# Autodesk Inventor assembly: daVinciHead_HITEC_Assembly
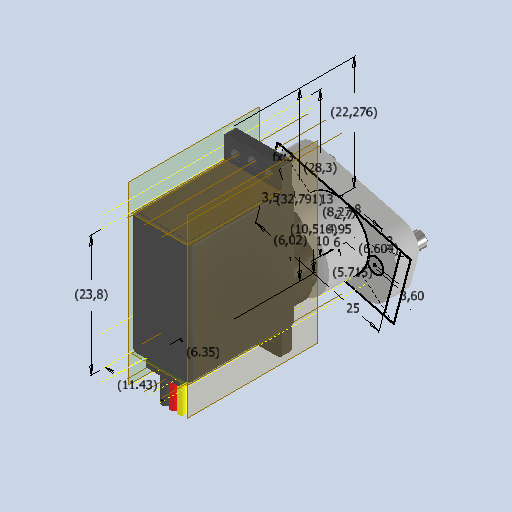
[picture p0: Inventor's stored thumbnail of the model, 512x512]
Saved by Autodesk Inventor 2024 (Build 280153000, 153)
## iProperties
Created: 2022-08-20
Part Number: daVinciHead_HITEC_Assembly
Document SubType Name: Assembly
Designer: alexw
Mass: 9.99183 g
Surface Area: 44.3615 cm^2
Volume: 8.83133 cm^3
Author: alexw
## Documents named in this file (6)
- C:\Users\AEWALDER\Documents\Inventor\03_CurrentProjects\MasterThesis\PSM_V1_Rillenkugellager\Ueberarbeiteter DaVincikopf\daVinciHead_HITEC_Assembly.iam
- C:\Users\AEWALDER\Documents\Inventor\03_CurrentProjects\MasterThesis\PSM_V1_Rillenkugellager\Ueberarbeiteter DaVincikopf\Hitec HS-65HB.ipt
- C:\Users\AEWALDER\Documents\Inventor\03_CurrentProjects\MasterThesis\PSM_V1_Rillenkugellager\Ueberarbeiteter DaVincikopf\daVinci_Tool_Clutch.ipt
- C:\Users\AEWALDER\Documents\Inventor\03_CurrentProjects\MasterThesis\PSM_V1_Rillenkugellager\Ueberarbeiteter DaVincikopf\daVinci_Tool_Clutch_Pins.ipt
- C:\Users\AEWALDER\Documents\Inventor\03_CurrentProjects\MasterThesis\PSM_V1_Rillenkugellager\ContentCenter\de-DE\ISO 4762(2)\ISO 4762 - M2 x 5ISO.ipt
- C:\Users\AEWALDER\Documents\Inventor\03_CurrentProjects\MasterThesis\PSM_V1_Rillenkugellager\ContentCenter\de-DE\ISO 7089\ISO 7089 - 2 - 140 HV(1).ipt
## Components (6 placed, 5 different names)
1. Hitec HS-65HB:1 — Fluchtend:1, Fluchtend:2, Fluchtend:3, Passend:7, Passend:11, Passend:12
2. daVinci_Tool_Clutch:1 — Passend:3, Passend:5, Passend:11, Passend:12, Fluchtend:4, Fluchtend:5, Passend:13
3. daVinci_Tool_Clutch_Pins:1 — Passend:3, Fluchtend:4
4. daVinci_Tool_Clutch_Pins:2 — Passend:5, Fluchtend:5
5. ISO 4762 M2 x 5:1 — Passend:7, Passend:8, Passend:10
6. ISO 7089 2:1 — Passend:8, Passend:10, Passend:13
## Relationships (13: Mate 8, Flush 5)
- Fluchtend:1 [Flush]: Hitec HS-65HB:1
- Fluchtend:2 [Flush]: Hitec HS-65HB:1
- Fluchtend:3 [Flush]: Hitec HS-65HB:1
- Passend:3 [Mate]: daVinci_Tool_Clutch:1 ↔ daVinci_Tool_Clutch_Pins:1
- Passend:5 [Mate]: daVinci_Tool_Clutch:1 ↔ daVinci_Tool_Clutch_Pins:2
- Passend:7 [Mate]: Hitec HS-65HB:1 ↔ ISO 4762 M2 x 5:1
- Passend:8 [Mate]: ISO 4762 M2 x 5:1 ↔ ISO 7089 2:1
- Passend:10 [Mate]: ISO 4762 M2 x 5:1 ↔ ISO 7089 2:1
- Passend:11 [Mate]: Hitec HS-65HB:1 ↔ daVinci_Tool_Clutch:1
- Passend:12 [Mate]: Hitec HS-65HB:1 ↔ daVinci_Tool_Clutch:1
- Fluchtend:4 [Flush]: daVinci_Tool_Clutch:1 ↔ daVinci_Tool_Clutch_Pins:1
- Fluchtend:5 [Flush]: daVinci_Tool_Clutch:1 ↔ daVinci_Tool_Clutch_Pins:2
- Passend:13 [Mate]: daVinci_Tool_Clutch:1 ↔ ISO 7089 2:1
